# Autodesk Inventor assembly: Circle_Cell
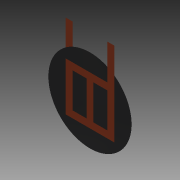
[picture p0: Inventor's stored thumbnail of the model, 180x180]
Saved by Autodesk Inventor 2014 SP1 (Build 180222100, 222)
## iProperties
Created: 2014-01-13
Part Number: Circle_Cell
Document SubType Name: Assembly
Designer: tuleu
Author: tuleu
## Documents named in this file (3)
- C:\Users\tuleu\Documents\giant-snes-gamepad\cad\Circle_Cell.iam
- C:\Users\tuleu\Documents\giant-snes-gamepad\cad\Circle_Velostat.ipt
- C:\Users\tuleu\Documents\giant-snes-gamepad\cad\Circle_Copper.ipt
## Components (3 placed, 2 different names)
1. Circle_Velostat:1 — Mate:1, Mate:2, Mate:3, Mate:4, Mate:5, Mate:6
2. Circle_Copper:1 — Mate:1, Mate:2, Mate:3
3. Circle_Copper:2 — Mate:4, Mate:5, Mate:6
## Relationships (6: Mate 6)
- Mate:1: Circle_Velostat:1 ↔ Circle_Copper:1
- Mate:2: Circle_Velostat:1 ↔ Circle_Copper:1
- Mate:3: Circle_Velostat:1 ↔ Circle_Copper:1
- Mate:4: Circle_Velostat:1 ↔ Circle_Copper:2
- Mate:5: Circle_Velostat:1 ↔ Circle_Copper:2
- Mate:6: Circle_Velostat:1 ↔ Circle_Copper:2
